# Autodesk Inventor assembly: 組合檔
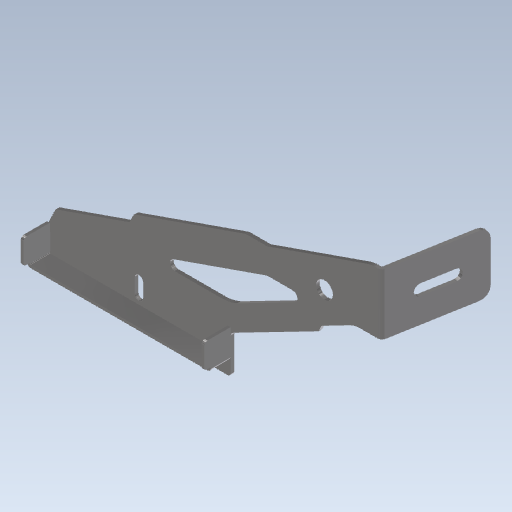
[picture p0: Inventor's stored thumbnail of the model, 512x512]
Saved by Autodesk Inventor 2020 (Build 240168000, 168)
## iProperties
Created: 2015-11-28
Part Number: 組合檔
Document SubType Name: Assembly
Designer: 設計製圖
Author: 設計製圖
## Documents named in this file (3)
- D:\資料庫\設計-3D Project\【May club 】\得利卡-車頂燈架\模型、圖面\22.01.05_設變 (未生產 )\吊架-短(R)(#01.05) - 焊接組合.iam
- D:\資料庫\設計-3D Project\【May club 】\得利卡-車頂燈架\模型、圖面\22.01.05_設變 (未生產 )\吊架-短(R)#01.05)- 焊接件-1.ipt
- D:\資料庫\設計-3D Project\【May club 】\得利卡-車頂燈架\模型、圖面\22.01.05_設變 (未生產 )\吊架-短(#01.05) - 焊接件-2.ipt
## Components (2 placed, 2 different names)
1. 吊架-短(R)#01.05)- 焊接件-1:1 — 貼合:1, 貼合:2, 貼合:3
2. 吊架-短(#01.05) - 焊接件-2:1 — 貼合:1, 貼合:2, 貼合:3
## Relationships (3: Mate 3)
- 貼合:1 [Mate]: 吊架-短(R)#01.05)- 焊接件-1:1 ↔ 吊架-短(#01.05) - 焊接件-2:1
- 貼合:2 [Mate]: 吊架-短(R)#01.05)- 焊接件-1:1 ↔ 吊架-短(#01.05) - 焊接件-2:1
- 貼合:3 [Mate]: 吊架-短(R)#01.05)- 焊接件-1:1 ↔ 吊架-短(#01.05) - 焊接件-2:1
